# Autodesk Inventor assembly: NameplateAsm
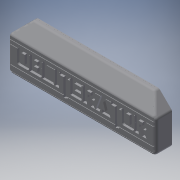
[picture p0: Inventor's stored thumbnail of the model, 180x180]
Saved by Autodesk Inventor 2018.3 (Build 223284000, 284)
## iProperties
Created: 2019-08-17
Part Number: NameplateAsm
Document SubType Name: Assembly
Designer: Srinity
Author: Srinity
## Documents named in this file (3)
- C:\Users\Srinity\Documents\DIY Projects\NerfGun\NameplateAsm.iam
- C:\Users\Srinity\Documents\DIY Projects\NerfGun\Nameplate.ipt
- C:\Users\Srinity\Documents\DIY Projects\NerfGun\Nameplatedrill.ipt
## Components (2 placed, 2 different names)
1. Nameplate:1 — Flush:1
2. Nameplatedrill:1 — Flush:1
## Relationships (1: Flush 1)
- Flush:1: Nameplate:1 ↔ Nameplatedrill:1
